# Autodesk Inventor assembly: HTR.B57B78B848E8AA1C977A1F7E292474E3
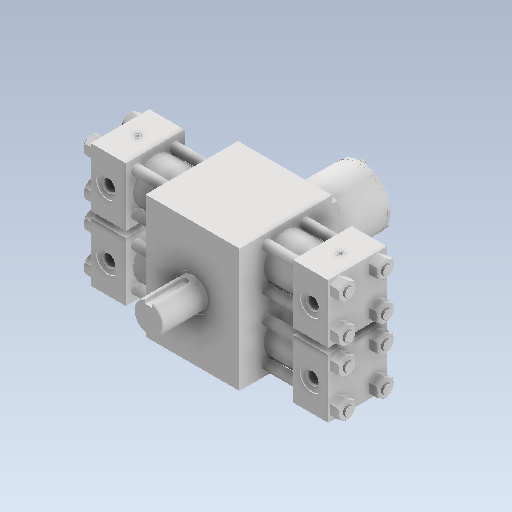
[picture p0: Inventor's stored thumbnail of the model, 512x512]
Saved by Autodesk Inventor 2021 (Build 250183000, 183)
## iProperties
Created: 2020-09-30
Part Number: HTR.B57B78B848E8AA1C977A1F7E292474E3
Document SubType Name: Assembly
Designer: InventorETOServices
Author: InventorETOServices
## Documents named in this file (4)
- D:\_\fctbqoxz5id0drsrkw3lze\Member Files\HTR.B57B78B848E8AA1C977A1F7E292474E3.iam
- D:\_\fctbqoxz5id0drsrkw3lze\Member Files\HTR7.5-INCHES.6B2CDF7C8F1732DD0B338AF01AA74AA6.ipt
- D:\_\fctbqoxz5id0drsrkw3lze\Member Files\ShaftConfig_B_3.7_7.5.FDA658ECE0FAA460A03A372F46ED1B09.ipt
- D:\_\fctbqoxz5id0drsrkw3lze\Member Files\HTR3.7-7.5_J+H.9E4C23B774108A62587442637768E7FC.ipt
## Components (3 placed, 3 different names)
1. Housing — AddConstraintHouseShaft, Mate_Shaft_Housing_Planes_1, Mate_Shaft_Housing_Axes_2, Mate_Shaft_Housing_Planes_3, Mate_Option_Housing_1, Mate_Option_Housing_2, Mate_Option_Housing_3
2. Shaft — AddConstraintHouseShaft, Mate_Shaft_Housing_Planes_1, Mate_Shaft_Housing_Axes_2, Mate_Shaft_Housing_Planes_3
3. options — Mate_Option_Housing_1, Mate_Option_Housing_2, Mate_Option_Housing_3
## Relationships (7: Mate 7)
- AddConstraintHouseShaft [Mate]: Housing ↔ Shaft
- Mate_Shaft_Housing_Planes_1: Housing ↔ Shaft
- Mate_Shaft_Housing_Axes_2: Housing ↔ Shaft
- Mate_Shaft_Housing_Planes_3: Housing ↔ Shaft
- Mate_Option_Housing_1: Housing ↔ options
- Mate_Option_Housing_2: Housing ↔ options
- Mate_Option_Housing_3: Housing ↔ options
